# Autodesk Inventor assembly: LiftPlate
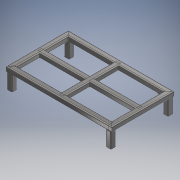
[picture p0: Inventor's stored thumbnail of the model, 180x180]
Saved by Autodesk Inventor 2018 (Build 220112000, 112)
## iProperties
Created: 2017-10-20
Part Number: LiftPlate
Document SubType Name: Weldment
Designer: Bryce Richards
Weld Material: Steel, Mild
Mass: 9609.17 g
Surface Area: 12362.4 cm^2
Volume: 1224.1 cm^3
Density: 7.85 g/cm^3
_SolveAssemblyDoc: Frame Generator Solve Assembly
_Version: 15.0.0
Author: Bryce Richards
## Documents named in this file (10)
- C:\Users\P136265\Documents\GitHub\mecanum-cad\LiftPlate.iam
- C:\Users\P136265\Documents\GitHub\mecanum-cad\LiftPlateWireframe.ipt
- C:\Users\P136265\Documents\GitHub\mecanum-cad\LiftPlate\Frame\Frame0001.iam
- C:\Users\P136265\Documents\GitHub\mecanum-cad\Gusset.ipt
- C:\Users\P136265\Documents\GitHub\mecanum-cad\LiftPlate\AIP\FEA\ciyzv7pxc.fins
- C:\Users\P136265\Documents\GitHub\mecanum-cad\LiftPlate\AIP\FEA\ciyzv7pxc.fsat
- C:\Users\P136265\Documents\GitHub\mecanum-cad\LiftPlate\AIP\FEA\ciyzv7pxc.ftes
- C:\Users\P136265\Documents\GitHub\mecanum-cad\LiftPlate\AIP\FEA\ciyzv7pxc.fwiz
- C:\Users\P136265\Documents\GitHub\mecanum-cad\LiftPlate\AIP\FEA\ciyzv7q2o.fmsh
- C:\Users\P136265\Documents\GitHub\mecanum-cad\LiftPlate\AIP\FEA\ciyzv7q2p.fres
## Components (3 placed, 3 different names)
1. LiftPlateWireframe:1
2. Frame0001:1 [sub-assembly] — Flush:1, Flush:2
3. Gusset:1 — Flush:1, Flush:2
## Relationships (2: Flush 2)
- Flush:1: Frame0001:1 ↔ Gusset:1
- Flush:2 (-17.5 mm): Frame0001:1 ↔ Gusset:1
## Named parameters: sa_0 = -1.05e-11, sa_1 = 0, sa_2 = 42500, sa_3 = -1.4e-11, sa_4 = 0, sa_5 = 42500
note: some values were not read from the file. Shown as the stored number, unit unknown: "sa_0", "sa_1", "sa_2", "sa_3", "sa_4", "sa_5".
